# Autodesk Inventor assembly: ComederoV3
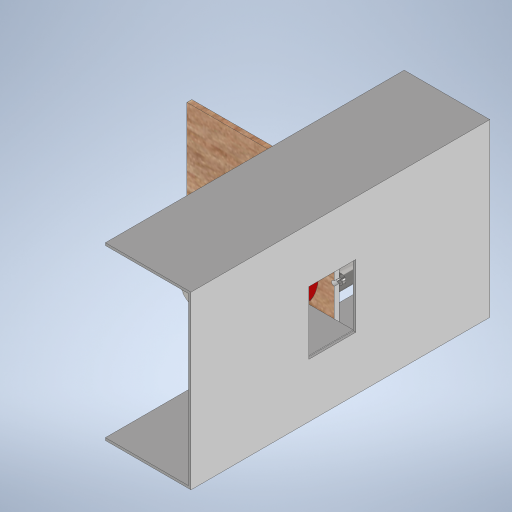
[picture p0: Inventor's stored thumbnail of the model, 512x512]
Saved by Autodesk Inventor 2023 (Build 270158000, 158)
## iProperties
Created: 2022-11-24
Part Number: ComederoV3
Document SubType Name: Assembly
Designer: sergi
Author: sergi
## Documents named in this file (9)
- C:\Users\sergi\OneDrive\Escritorio\Objetos 3d\ComederoV2\ComederoV3.iam
- C:\Users\sergi\OneDrive\Escritorio\Objetos 3d\ComederoV2\Camisa.ipt
- C:\Users\sergi\OneDrive\Escritorio\Objetos 3d\ComederoV2\Embudo.ipt
- C:\Users\sergi\OneDrive\Escritorio\Objetos 3d\ComederoV2\Plataforma.ipt
- C:\Users\sergi\OneDrive\Escritorio\Objetos 3d\ComederoV2\Rampa.ipt
- C:\Users\sergi\OneDrive\Escritorio\Objetos 3d\ComederoV2\Caja.ipt
- C:\Users\sergi\OneDrive\Escritorio\Objetos 3d\ComederoV2\ComederoV3\Design Accelerator\Engranajes helicoidales2.iam
- C:\Users\sergi\OneDrive\Escritorio\Objetos 3d\ComederoV2\Rampa2.ipt
- C:\Users\sergi\OneDrive\Escritorio\Objetos 3d\ComederoV2\Barra M8.ipt
## Components (8 placed, 8 different names)
1. Camisa:1
2. Embudo:1 — Coincidencia:2
3. Plataforma:1 — Coincidencia:3
4. Rampa:1
5. Caja:1
6. Engranajes helicoidales:1 [sub-assembly] — Nivelación:1, Coincidencia:1
7. Rampa2:1
8. Barra M8:1 — Nivelación:1, Coincidencia:1, Coincidencia:2, Coincidencia:3
## Relationships (4: Mate 3, Flush 1)
- Nivelación:1 [Flush]: Engranajes helicoidales:1 ↔ Barra M8:1
- Coincidencia:1 [Mate]: Engranajes helicoidales:1 ↔ Barra M8:1
- Coincidencia:2 [Mate]: Embudo:1 ↔ Barra M8:1
- Coincidencia:3 [Mate]: Plataforma:1 ↔ Barra M8:1
